# Autodesk Inventor assembly: MotorFilamentSpool
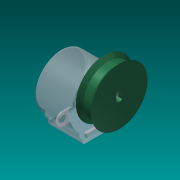
[picture p0: Inventor's stored thumbnail of the model, 180x180]
Saved by Autodesk Inventor 2013 (Build 170138000, 138)
## iProperties
Created: 2013-08-16
Part Number: MotorFilamentSpool
Document SubType Name: Assembly
Designer: Sawaiz
Author: Sawaiz
## Documents named in this file (3)
- S:\Sawaiz\Documents\3D Modeling\Inventor\PolarGraph\MotorFilamentSpool.iam
- S:\Sawaiz\Documents\3D Modeling\Inventor\PolarGraph\Stepper Motor 28BYJ-48.ipt
- S:\Sawaiz\Documents\3D Modeling\Inventor\PolarGraph\MonoFilamentSpool.iam
## Components (2 placed, 2 different names)
1. Stepper Motor 28BYJ-48:1 — Mate:1, Flush:1
2. MonoFilamentSpool:1 [sub-assembly] — Mate:1, Flush:1
## Relationships (2: Mate 1, Flush 1)
- Mate:1: Stepper Motor 28BYJ-48:1 ↔ MonoFilamentSpool:1
- Flush:1: Stepper Motor 28BYJ-48:1 ↔ MonoFilamentSpool:1
